# Autodesk Inventor assembly: 組合檔
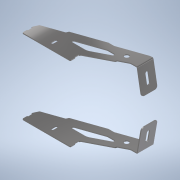
[picture p0: Inventor's stored thumbnail of the model, 180x180]
Saved by Autodesk Inventor 2020 (Build 240168000, 168)
## iProperties
Created: 2015-11-28
Part Number: 組合檔
Document SubType Name: Assembly
Designer: 設計製圖
Author: 設計製圖
## Documents named in this file (3)
- D:\資料庫\設計-3D Project\【May club 】\得利卡-車頂燈架\模型、圖面\短-車頂燈架-組合(#01.05)\鏡射用--吊架-短(R)#01.05)- 焊接件-1.iam
- D:\資料庫\設計-3D Project\【May club 】\得利卡-車頂燈架\模型、圖面\短-車頂燈架-組合(#01.05)\吊架-短(R)#01.05)- 焊接件-1.ipt
- D:\資料庫\設計-3D Project\【May club 】\得利卡-車頂燈架\模型、圖面\短-車頂燈架-組合(#01.05)\吊架-短(L)#01.05)- 焊接件-1_MIR.ipt
## Components (2 placed, 2 different names)
1. 吊架-短(R)#01.05)- 焊接件-1:1 — 齊平:1
2. 吊架-短(L)#01.05)- 焊接件-1_MIR:1 — 貼合:1
## Relationships (2: Flush 1, Mate 1)
- 齊平:1 [Flush] (100 mm): 吊架-短(R)#01.05)- 焊接件-1:1
- 貼合:1 [Mate] (100 mm): 吊架-短(L)#01.05)- 焊接件-1_MIR:1
